# Autodesk Inventor assembly: Assembly10
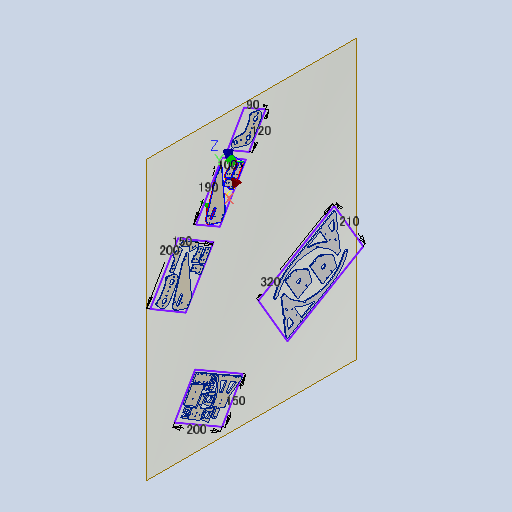
[picture p0: Inventor's stored thumbnail of the model, 512x512]
Saved by Autodesk Inventor 2025.2 (Build 292293000, 293)
## iProperties
Created: 2025-03-13
Part Number: Assembly10
Document SubType Name: Assembly
Designer: haruy
Author: haruy
## Documents named in this file (16)
- C:\Users\haruy\Documents\ロボコン\NHK2025\cad\cnc\Assembly10.iam
- C:\Users\haruy\Documents\ロボコン\NHK2025\cad\nagahisa\belt_liner\belt_liner_v5_Plate_7.ipt
- C:\Users\haruy\Documents\ロボコン\NHK2025\cad\nagahisa\belt_liner\belt_liner_v5_Plate_1.ipt
- C:\Users\haruy\Documents\ロボコン\NHK2025\cad\nagahisa\belt_liner\belt_liner_v5_Plate_8.ipt
- C:\Users\haruy\Documents\ロボコン\NHK2025\cad\nagahisa\belt_liner\belt_liner_v5_Plate_11.ipt
- C:\Users\haruy\Documents\ロボコン\NHK2025\cad\nagahisa\belt_liner\belt_liner_v5_Plate_9.ipt
- C:\Users\haruy\Documents\ロボコン\NHK2025\cad\nagahisa\belt_liner\belt_liner_v5_Plate_3.ipt
- C:\Users\haruy\Documents\ロボコン\NHK2025\cad\nagahisa\belt_liner\belt_liner_v5_Plate_2.ipt
- C:\Users\haruy\Documents\ロボコン\NHK2025\cad\nagahisa\belt_liner\belt_liner_v5_Plate_10.ipt
- C:\Users\haruy\Documents\ロボコン\NHK2025\cad\nagahisa\belt_liner\belt_liner_v5_Plate_5.ipt
- C:\Users\haruy\Documents\ロボコン\NHK2025\cad\nagahisa\belt_liner\belt_liner_v5_Plate_12.ipt
- C:\Users\haruy\Documents\ロボコン\NHK2025\cad\nagahisa\belt_liner\belt_liner_v5_Plate_6.ipt
- C:\Users\haruy\Documents\ロボコン\NHK2025\cad\nagahisa\belt_liner\belt_liner_v5_Plate_16.ipt
- C:\Users\haruy\Documents\ロボコン\NHK2025\cad\nagahisa\belt_liner\belt_liner_v5_Plate_15.ipt
- C:\Users\haruy\Documents\ロボコン\NHK2025\cad\nagahisa\belt_liner\belt_liner_v5_Plate_14.ipt
- C:\Users\haruy\Documents\ロボコン\NHK2025\cad\nagahisa\dribl\dribl-v1-Plate-14.ipt
## Components (28 placed, 15 different names)
1. belt_liner_v5_Plate_7:1 — メイト:1, フラッシュ:1, 角度:1, フラッシュ:2, 角度:2, 角度:3
2. belt_liner_v5_Plate_7:2 — フラッシュ:1, 角度:1
3. belt_liner_v5_Plate_1:1 — フラッシュ:2, フラッシュ:3, 角度:2
4. belt_liner_v5_Plate_1:2 — フラッシュ:3, 角度:3
5. belt_liner_v5_Plate_8:1 — フラッシュ:4, フラッシュ:5, フラッシュ:9, フラッシュ:10, フラッシュ:13, メイト:6, フラッシュ:14, フラッシュ:19, メイト:11, メイト:13
6. belt_liner_v5_Plate_11:1 — フラッシュ:5, フラッシュ:6, メイト:3, フラッシュ:8, メイト:16, メイト:17
7. belt_liner_v5_Plate_11:2 — フラッシュ:6, メイト:3, フラッシュ:8
8. belt_liner_v5_Plate_9:1 — フラッシュ:9, フラッシュ:10, フラッシュ:11, メイト:5, フラッシュ:12, メイト:11
9. belt_liner_v5_Plate_9:2 — フラッシュ:11, メイト:5, フラッシュ:12, メイト:12
10. belt_liner_v5_Plate_3:1 — フラッシュ:13, メイト:6, フラッシュ:14, フラッシュ:15, フラッシュ:16, メイト:8, フラッシュ:18, メイト:14, メイト:15, メイト:16, フラッシュ:21
11. belt_liner_v5_Plate_2:1 — フラッシュ:15, メイト:14, メイト:15, メイト:17, フラッシュ:22
12. belt_liner_v5_Plate_10:1 — フラッシュ:16, メイト:8, フラッシュ:17, メイト:10, メイト:13, フラッシュ:20
13. belt_liner_v5_Plate_10:2 — フラッシュ:17, メイト:10, フラッシュ:20
14. belt_liner_v5_Plate_5:1 — フラッシュ:18, フラッシュ:19, メイト:12
15. belt_liner_v5_Plate_12:1 — フラッシュ:21
16. belt_liner_v5_Plate_12:2 — フラッシュ:22
17. belt_liner_v5_Plate_6:1 — フラッシュ:23, フラッシュ:24, フラッシュ:26, フラッシュ:29, 角度:7, フラッシュ:34, フラッシュ:36
18. belt_liner_v5_Plate_16:1 — フラッシュ:24, 角度:7
19. belt_liner_v5_Plate_16:2 — フラッシュ:34, 角度:8
20. belt_liner_v5_Plate_15:1 — フラッシュ:26, フラッシュ:27, フラッシュ:28, 角度:5
21. belt_liner_v5_Plate_14:1 — フラッシュ:27, フラッシュ:43
22. dribl-v1-Plate-14:1 — フラッシュ:28, フラッシュ:29, フラッシュ:30, フラッシュ:31, フラッシュ:32, メイト:19
23. dribl-v1-Plate-14:2 — フラッシュ:30, メイト:18, フラッシュ:33, 角度:8
24. dribl-v1-Plate-14:3 — フラッシュ:31, フラッシュ:32, メイト:18, フラッシュ:33, メイト:19, 角度:5, フラッシュ:35
25. belt_liner_v5_Plate_6:2 — フラッシュ:35, フラッシュ:36, フラッシュ:37, フラッシュ:38, フラッシュ:40
26. dribl-v1-Plate-14:4 — フラッシュ:37, メイト:20, フラッシュ:39, フラッシュ:40, フラッシュ:43
27. dribl-v1-Plate-14:5 — フラッシュ:38, メイト:20, フラッシュ:39, フラッシュ:41, メイト:21, フラッシュ:42
28. dribl-v1-Plate-14:6 — フラッシュ:41, メイト:21, フラッシュ:42
## Relationships (64: Flush 41, Mate 17, Angle 6)
- メイト:1 [Mate]: belt_liner_v5_Plate_7:1
- フラッシュ:1 [Flush]: belt_liner_v5_Plate_7:1 ↔ belt_liner_v5_Plate_7:2
- 角度:1 [Angle] (180 deg): belt_liner_v5_Plate_7:1 ↔ belt_liner_v5_Plate_7:2
- フラッシュ:2 [Flush]: belt_liner_v5_Plate_7:1 ↔ belt_liner_v5_Plate_1:1
- フラッシュ:3 [Flush]: belt_liner_v5_Plate_1:1 ↔ belt_liner_v5_Plate_1:2
- 角度:2 [Angle] (0 deg): belt_liner_v5_Plate_7:1 ↔ belt_liner_v5_Plate_1:1
- 角度:3 [Angle] (0 deg): belt_liner_v5_Plate_7:1 ↔ belt_liner_v5_Plate_1:2
- フラッシュ:4 [Flush]: belt_liner_v5_Plate_8:1
- フラッシュ:5 [Flush]: belt_liner_v5_Plate_8:1 ↔ belt_liner_v5_Plate_11:1
- フラッシュ:6 [Flush]: belt_liner_v5_Plate_11:1 ↔ belt_liner_v5_Plate_11:2
- メイト:3 [Mate] (5 mm): belt_liner_v5_Plate_11:1 ↔ belt_liner_v5_Plate_11:2
- フラッシュ:8 [Flush]: belt_liner_v5_Plate_11:1 ↔ belt_liner_v5_Plate_11:2
- フラッシュ:9 [Flush]: belt_liner_v5_Plate_8:1 ↔ belt_liner_v5_Plate_9:1
- フラッシュ:10 [Flush]: belt_liner_v5_Plate_8:1 ↔ belt_liner_v5_Plate_9:1
- フラッシュ:11 [Flush]: belt_liner_v5_Plate_9:1 ↔ belt_liner_v5_Plate_9:2
- メイト:5 [Mate] (5 mm): belt_liner_v5_Plate_9:1 ↔ belt_liner_v5_Plate_9:2
- フラッシュ:12 [Flush]: belt_liner_v5_Plate_9:1 ↔ belt_liner_v5_Plate_9:2
- フラッシュ:13 [Flush]: belt_liner_v5_Plate_8:1 ↔ belt_liner_v5_Plate_3:1
- メイト:6 [Mate] (5 mm): belt_liner_v5_Plate_8:1 ↔ belt_liner_v5_Plate_3:1
- フラッシュ:14 [Flush]: belt_liner_v5_Plate_8:1 ↔ belt_liner_v5_Plate_3:1
- フラッシュ:15 [Flush]: belt_liner_v5_Plate_3:1 ↔ belt_liner_v5_Plate_2:1
- フラッシュ:16 [Flush]: belt_liner_v5_Plate_3:1 ↔ belt_liner_v5_Plate_10:1
- メイト:8 [Mate] (5 mm): belt_liner_v5_Plate_3:1 ↔ belt_liner_v5_Plate_10:1
- フラッシュ:17 [Flush]: belt_liner_v5_Plate_10:1 ↔ belt_liner_v5_Plate_10:2
- メイト:10 [Mate] (5 mm): belt_liner_v5_Plate_10:1 ↔ belt_liner_v5_Plate_10:2
- フラッシュ:18 [Flush]: belt_liner_v5_Plate_3:1 ↔ belt_liner_v5_Plate_5:1
- フラッシュ:19 [Flush]: belt_liner_v5_Plate_8:1 ↔ belt_liner_v5_Plate_5:1
- メイト:11 [Mate] (5 mm): belt_liner_v5_Plate_8:1 ↔ belt_liner_v5_Plate_9:1
- メイト:12 [Mate] (5 mm): belt_liner_v5_Plate_9:2 ↔ belt_liner_v5_Plate_5:1
- メイト:13 [Mate] (5 mm): belt_liner_v5_Plate_8:1 ↔ belt_liner_v5_Plate_10:1
- フラッシュ:20 [Flush]: belt_liner_v5_Plate_10:1 ↔ belt_liner_v5_Plate_10:2
- メイト:14 [Mate] (5 mm): belt_liner_v5_Plate_3:1 ↔ belt_liner_v5_Plate_2:1
- メイト:15 [Mate] (5 mm): belt_liner_v5_Plate_3:1 ↔ belt_liner_v5_Plate_2:1
- メイト:16 [Mate] (5 mm): belt_liner_v5_Plate_11:1 ↔ belt_liner_v5_Plate_3:1
- メイト:17 [Mate] (5 mm): belt_liner_v5_Plate_11:1 ↔ belt_liner_v5_Plate_2:1
- フラッシュ:21 [Flush]: belt_liner_v5_Plate_3:1 ↔ belt_liner_v5_Plate_12:1
- フラッシュ:22 [Flush]: belt_liner_v5_Plate_2:1 ↔ belt_liner_v5_Plate_12:2
- フラッシュ:23 [Flush]: belt_liner_v5_Plate_6:1
- フラッシュ:24 [Flush]: belt_liner_v5_Plate_6:1 ↔ belt_liner_v5_Plate_16:1
- フラッシュ:26 [Flush]: belt_liner_v5_Plate_6:1 ↔ belt_liner_v5_Plate_15:1
- フラッシュ:27 [Flush]: belt_liner_v5_Plate_15:1 ↔ belt_liner_v5_Plate_14:1
- フラッシュ:28 [Flush]: belt_liner_v5_Plate_15:1 ↔ dribl-v1-Plate-14:1
- フラッシュ:29 [Flush]: belt_liner_v5_Plate_6:1 ↔ dribl-v1-Plate-14:1
- フラッシュ:30 [Flush]: dribl-v1-Plate-14:1 ↔ dribl-v1-Plate-14:2
- フラッシュ:31 [Flush]: dribl-v1-Plate-14:1 ↔ dribl-v1-Plate-14:3
- フラッシュ:32 [Flush]: dribl-v1-Plate-14:1 ↔ dribl-v1-Plate-14:3
- メイト:18 [Mate] (5 mm): dribl-v1-Plate-14:2 ↔ dribl-v1-Plate-14:3
- フラッシュ:33 [Flush]: dribl-v1-Plate-14:2 ↔ dribl-v1-Plate-14:3
- メイト:19 [Mate] (5 mm): dribl-v1-Plate-14:1 ↔ dribl-v1-Plate-14:3
- 角度:5 [Angle] (0 deg): belt_liner_v5_Plate_15:1 ↔ dribl-v1-Plate-14:3
- 角度:7 [Angle] (180 deg): belt_liner_v5_Plate_6:1 ↔ belt_liner_v5_Plate_16:1
- フラッシュ:34 [Flush]: belt_liner_v5_Plate_6:1 ↔ belt_liner_v5_Plate_16:2
- 角度:8 [Angle] (210 deg): belt_liner_v5_Plate_16:2 ↔ dribl-v1-Plate-14:2
- フラッシュ:35 [Flush]: dribl-v1-Plate-14:3 ↔ belt_liner_v5_Plate_6:2
- フラッシュ:36 [Flush]: belt_liner_v5_Plate_6:1 ↔ belt_liner_v5_Plate_6:2
- フラッシュ:37 [Flush]: belt_liner_v5_Plate_6:2 ↔ dribl-v1-Plate-14:4
- フラッシュ:38 [Flush]: belt_liner_v5_Plate_6:2 ↔ dribl-v1-Plate-14:5
- メイト:20 [Mate] (5 mm): dribl-v1-Plate-14:4 ↔ dribl-v1-Plate-14:5
- フラッシュ:39 [Flush]: dribl-v1-Plate-14:4 ↔ dribl-v1-Plate-14:5
- フラッシュ:40 [Flush]: belt_liner_v5_Plate_6:2 ↔ dribl-v1-Plate-14:4
- フラッシュ:41 [Flush]: dribl-v1-Plate-14:5 ↔ dribl-v1-Plate-14:6
- メイト:21 [Mate] (5 mm): dribl-v1-Plate-14:5 ↔ dribl-v1-Plate-14:6
- フラッシュ:42 [Flush]: dribl-v1-Plate-14:5 ↔ dribl-v1-Plate-14:6
- フラッシュ:43 [Flush]: belt_liner_v5_Plate_14:1 ↔ dribl-v1-Plate-14:4
